# Autodesk Inventor assembly: A4988_driver-asm
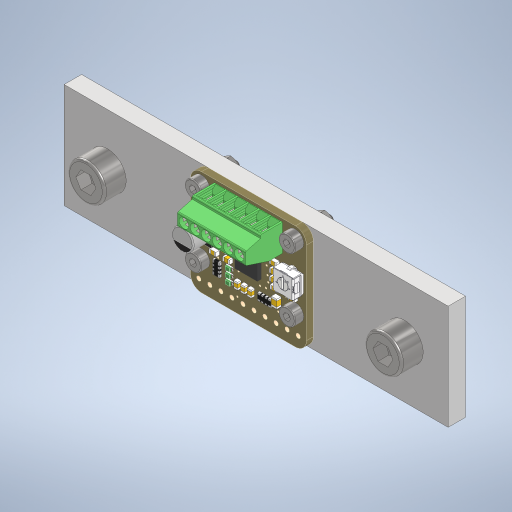
[picture p0: Inventor's stored thumbnail of the model, 512x512]
Saved by Autodesk Inventor 2024 (Build 280153000, 153)
## iProperties
Created: 2026-01-01
Part Number: A4988_driver-asm
Document SubType Name: Assembly
Designer: schar
Author: schar
## Documents named in this file (7)
- C:\Users\schar\Desktop\projectBlueprint\AMSTS\hardware\A4988_driver-asm.iam
- C:\Users\schar\Desktop\projectBlueprint\AMSTS\hardware\A4988_driver_hodler.ipt
- C:\Users\schar\Desktop\projectBlueprint\AMSTS\hardware\6109 A4988 Driver.iam
- C:\Users\schar\Documents\Inventor\Content Center Files\R2024\en-US\ISO 4762(1)\DIN EN ISO 4762 - M2 x 8.ipt
- C:\Users\schar\Desktop\projectBlueprint\AMSTS\hardware\tnut_m5_2020.ipt
- C:\Users\schar\Documents\Inventor\Content Center Files\R2024\en-US\DIN EN ISO 4032\DIN EN ISO 4032 - M2.ipt
- C:\Users\schar\Documents\Inventor\Content Center Files\R2024\en-US\ISO 4762(1)\DIN EN ISO 4762 - M5 x 10.ipt
## Components (14 placed, 6 different names)
1. A4988_driver_hodler:1 — Mate:1, Mate:2, Mate:3, Mate:8, Mate:9, Mate:10, Mate:11, Rigid:1, Rigid:2, Mate:12, Mate:13, Mate:14, Mate:15, Mate:20, Mate:21
2. 6109 A4988 Driver:1 [sub-assembly] — Mate:1, Mate:2, Mate:3, Mate:4, Mate:5, Mate:6, Mate:7
3. DIN EN ISO 4762 M2 x 8:1 — Mate:7, Mate:9, Mate:18
4. DIN EN ISO 4762 M2 x 8:2 — Mate:6, Mate:8, Mate:17
5. DIN EN ISO 4762 M2 x 8:3 — Mate:5, Mate:10, Mate:16
6. DIN EN ISO 4762 M2 x 8:4 — Mate:4, Mate:11, Mate:19
7. tnut_m5_2020:1 — Rigid:1, Mate:23
8. tnut_m5_2020:2 — Rigid:2, Mate:22
9. DIN EN ISO 4032 M2:1 — Mate:14, Mate:18
10. DIN EN ISO 4032 M2:2 — Mate:15, Mate:16
11. DIN EN ISO 4032 M2:3 — Mate:13, Mate:17
12. DIN EN ISO 4032 M2:4 — Mate:12, Mate:19
13. DIN EN ISO 4762 M5 x 10:1 — Mate:21, Mate:22
14. DIN EN ISO 4762 M5 x 10:2 — Mate:20, Mate:23
## Relationships (25: Mate 23, WeldJoint 2)
- Mate:1: A4988_driver_hodler:1 ↔ 6109 A4988 Driver:1
- Mate:2: A4988_driver_hodler:1 ↔ 6109 A4988 Driver:1
- Mate:3: A4988_driver_hodler:1 ↔ 6109 A4988 Driver:1
- Mate:4: 6109 A4988 Driver:1 ↔ DIN EN ISO 4762 M2 x 8:4
- Mate:5: 6109 A4988 Driver:1 ↔ DIN EN ISO 4762 M2 x 8:3
- Mate:6: 6109 A4988 Driver:1 ↔ DIN EN ISO 4762 M2 x 8:2
- Mate:7: 6109 A4988 Driver:1 ↔ DIN EN ISO 4762 M2 x 8:1
- Mate:8: A4988_driver_hodler:1 ↔ DIN EN ISO 4762 M2 x 8:2
- Mate:9: A4988_driver_hodler:1 ↔ DIN EN ISO 4762 M2 x 8:1
- Mate:10: A4988_driver_hodler:1 ↔ DIN EN ISO 4762 M2 x 8:3
- Mate:11: A4988_driver_hodler:1 ↔ DIN EN ISO 4762 M2 x 8:4
- Rigid:1 [WeldJoint] (-0.159 mm): A4988_driver_hodler:1 ↔ tnut_m5_2020:1
- Rigid:2 [WeldJoint] (-0.159 mm): A4988_driver_hodler:1 ↔ tnut_m5_2020:2
- Mate:12: A4988_driver_hodler:1 ↔ DIN EN ISO 4032 M2:4
- Mate:13: A4988_driver_hodler:1 ↔ DIN EN ISO 4032 M2:3
- Mate:14: A4988_driver_hodler:1 ↔ DIN EN ISO 4032 M2:1
- Mate:15: A4988_driver_hodler:1 ↔ DIN EN ISO 4032 M2:2
- Mate:16: DIN EN ISO 4762 M2 x 8:3 ↔ DIN EN ISO 4032 M2:2
- Mate:17: DIN EN ISO 4762 M2 x 8:2 ↔ DIN EN ISO 4032 M2:3
- Mate:18: DIN EN ISO 4762 M2 x 8:1 ↔ DIN EN ISO 4032 M2:1
- Mate:19: DIN EN ISO 4762 M2 x 8:4 ↔ DIN EN ISO 4032 M2:4
- Mate:20: A4988_driver_hodler:1 ↔ DIN EN ISO 4762 M5 x 10:2
- Mate:21: A4988_driver_hodler:1 ↔ DIN EN ISO 4762 M5 x 10:1
- Mate:22: tnut_m5_2020:2 ↔ DIN EN ISO 4762 M5 x 10:1
- Mate:23: tnut_m5_2020:1 ↔ DIN EN ISO 4762 M5 x 10:2
